# Autodesk Inventor assembly: openFrame - explodable 5
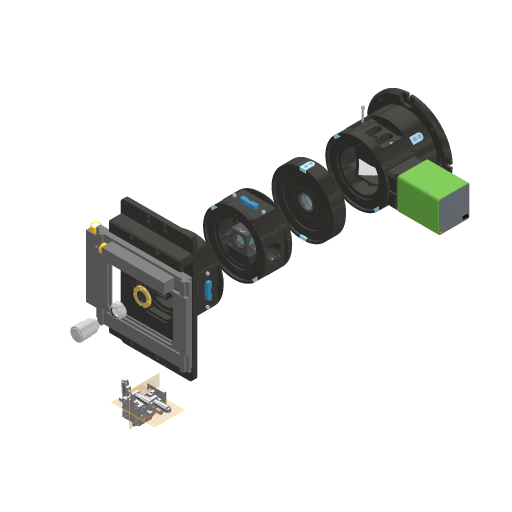
[picture p0: Inventor's stored thumbnail of the model, 512x512]
Saved by Autodesk Inventor 2024.1 (Build 281209000, 209)
## iProperties
Created: 2024-05-24
Part Number: openFrame - explodable 5
Description: STEP AP242
Document SubType Name: Assembly
Designer: diederichbenedict
Preprocessor: ST-DEVELOPER v20
Title: 664a3059de469d2f43417ff2
## Documents named in this file (15)
- C:\Users\diederichbenedict\Dropbox\Dokumente\Promotion\PROJECTS\SIMMO\INVENTOR\00_openFrameExplodable5\00_openFrameExplodable5.iam
- C:\Users\diederichbenedict\Dropbox\Dokumente\Promotion\PROJECTS\SIMMO\INVENTOR\00_openFrameExplodable5\OpenFrame - Stage Adapter.ipt
- C:\Users\diederichbenedict\Dropbox\Dokumente\Promotion\PROJECTS\SIMMO\INVENTOR\00_openFrameExplodable5\Part 1.ipt
- C:\Users\diederichbenedict\Dropbox\Dokumente\Promotion\PROJECTS\SIMMO\INVENTOR\00_openFrameExplodable5\OpenFrame - Objective Disc.ipt
- C:\Users\diederichbenedict\Dropbox\Dokumente\Promotion\PROJECTS\SIMMO\INVENTOR\00_openFrameExplodable5\Zaber Stage Risers - Piezo.ipt
- C:\Users\diederichbenedict\Dropbox\Dokumente\Promotion\PROJECTS\SIMMO\INVENTOR\00_openFrameExplodable5\OpenFrame - Olympus Objective Adapter.ipt
- C:\Users\diederichbenedict\Dropbox\Dokumente\Promotion\PROJECTS\SIMMO\INVENTOR\00_openFrameExplodable5\OF-LL-BP _1_.iam
- C:\Users\diederichbenedict\Dropbox\Dokumente\Promotion\PROJECTS\SIMMO\INVENTOR\00_openFrameExplodable5\OpenFrame - Camera C-Mount Coupling - 60mm Cage Version.ipt
- C:\Users\diederichbenedict\Dropbox\Dokumente\Promotion\PROJECTS\SIMMO\INVENTOR\00_openFrameExplodable5\Standin camera _1_.iam
- C:\Users\diederichbenedict\Dropbox\Dokumente\Promotion\PROJECTS\SIMMO\INVENTOR\00_openFrameExplodable5\OF-LL-TL - populated _1_.iam
- C:\Users\diederichbenedict\Dropbox\Dokumente\Promotion\PROJECTS\SIMMO\INVENTOR\00_openFrameExplodable5\Stage_assembly _1_.iam
- C:\Users\diederichbenedict\Dropbox\Dokumente\Promotion\PROJECTS\SIMMO\INVENTOR\00_openFrameExplodable5\OF-LL-FL-MOT - populated unmated _1_.iam
- C:\Users\diederichbenedict\Dropbox\Dokumente\Promotion\PROJECTS\SIMMO\INVENTOR\00_openFrameExplodable5\OF-LL-80 populated - MCH M45 unmated _1_.iam
- C:\Users\diederichbenedict\Dropbox\Dokumente\Promotion\PROJECTS\SIMMO\INVENTOR\00_openFrameExplodable5\OF-LL-65 - populated mated _1_.iam
- C:\Users\diederichbenedict\Dropbox\Dokumente\Promotion\PROJECTS\SIMMO\INVENTOR\00_openFrameExplodable5\00_XYZstage_micro_LT-4047-S1.ipt
## Components (15 placed, 15 different names)
1. NAUO1
2. NAUO2
3. NAUO3
4. NAUO4
5. NAUO5
6. NAUO6
7. NAUO19 [sub-assembly] — Einfügen:1, Winkel:1
8. NAUO20
9. NAUO27 [sub-assembly]
10. NAUO44 [sub-assembly]
11. NAUO54 [sub-assembly]
12. NAUO106 [sub-assembly]
13. NAUO148 [sub-assembly] — Einfügen:1, Winkel:1
14. NAUO199 [sub-assembly]
15. 00_XYZstage_micro_LT-4047-S1:1
## Relationships (2: Insert 1, Angle 1)
- Einfügen:1 [Insert]: NAUO19 ↔ NAUO148
- Winkel:1 [Angle] (269.8631 deg): NAUO19 ↔ NAUO148
